# Autodesk Inventor assembly: outer_mirrored
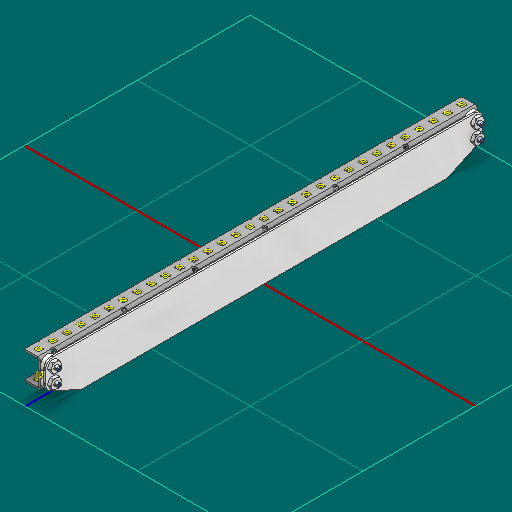
[picture p0: Inventor's stored thumbnail of the model, 512x512]
Saved by Autodesk Inventor 2025 (Build 290162000, 162)
## iProperties
Created: 2024-08-21
Part Number: outer_mirrored
Document SubType Name: Assembly
Designer: averey
Author: averey
## Documents named in this file (10)
- C:\Users\avere\vex_robotics_high_stakes\hardware\cad\bots\ENIGMA\chassis\drivetrain\drivebay_mirrored\outer_mirrored.iam
- C:\Users\avere\vex_robotics_high_stakes\hardware\cad\bots\ENIGMA\chassis\drivetrain\drivebay_mirrored\Alu C 1x2x1x31_mirrored.ipt
- C:\Users\avere\vex_robotics_high_stakes\hardware\cad\bots\ENIGMA\chassis\drivetrain\drivebay_mirrored\bearing_flat_w_hardware_mirrored.iam
- C:\Users\avere\vex_robotics_high_stakes\hardware\cad\VEX-CAD-Inventor\Motion\Spacers\Spacer Nylon .500 OD\NSpacer White .500 OD x .125.ipt
- C:\Users\avere\vex_robotics_high_stakes\hardware\cad\VEX-CAD-Inventor\Motion\Spacers\Spacer Nylon .500 OD.ipt
- C:\Users\avere\vex_robotics_high_stakes\hardware\cad\bots\ENIGMA\chassis\drivetrain\drivebay\custom_parts\skirt.ipt
- C:\Users\avere\vex_robotics_high_stakes\hardware\cad\VEX-CAD-Inventor\Structure\Hardware\Screw Shoulder Robosource\SScrew Shoulder Smooth .500 x .04.ipt
- C:\Users\avere\vex_robotics_high_stakes\hardware\cad\VEX-CAD-Inventor\Structure\Hardware\Screw Shoulder Robosource.ipt
- C:\Users\avere\vex_robotics_high_stakes\hardware\cad\VEX-CAD-Inventor\Structure\Hardware\Nut Nylon\Nut Nylon - White.ipt
- C:\Users\avere\vex_robotics_high_stakes\hardware\cad\VEX-CAD-Inventor\Structure\Hardware\Nut Nylon.ipt
## Components (23 placed, 6 different names)
1. Alu C 1x2x1x31_mirrored:1 — Mate:2, Mate:1, Mate:3, Insert:1, Insert:2, Insert:4
2. skirt:1 — Insert:3, Insert:5
3. bearing_flat_w_hardware_mirrored:1 [sub-assembly] — Mate:3, Insert:1
4. bearing_flat_w_hardware_mirrored:2 [sub-assembly]
5. bearing_flat_w_hardware_mirrored:3 [sub-assembly]
6. bearing_flat_w_hardware_mirrored:4 [sub-assembly]
7. bearing_flat_w_hardware_mirrored:5 [sub-assembly]
8. bearing_flat_w_hardware_mirrored:6 [sub-assembly]
9. bearing_flat_w_hardware_mirrored:7 [sub-assembly]
10. bearing_flat_w_hardware_mirrored:8 [sub-assembly]
11. bearing_flat_w_hardware_mirrored:9 [sub-assembly]
12. Nut Nylon - White:1 — Insert:5
13. SScrew Shoulder Smooth .500 x .04:1 — Insert:4
14. NSpacer White .500 OD x .125:1 — Insert:2, Insert:3
15. Nut Nylon - White:2
16. SScrew Shoulder Smooth .500 x .04:2
17. NSpacer White .500 OD x .125:2
18. Nut Nylon - White:3
19. SScrew Shoulder Smooth .500 x .04:3
20. NSpacer White .500 OD x .125:3
21. Nut Nylon - White:4
22. SScrew Shoulder Smooth .500 x .04:4
23. NSpacer White .500 OD x .125:4
## Component patterns: (9 elements, first: bearing_flat_w_hardware_mirrored:1), Hardware (4 elements)
## Relationships (8: Insert 5, Mate 3)
- Mate:2 (11.1125 mm): Alu C 1x2x1x31_mirrored:1
- Mate:1: Alu C 1x2x1x31_mirrored:1
- Mate:3: Alu C 1x2x1x31_mirrored:1 ↔ bearing_flat_w_hardware_mirrored:1
- Insert:1: Alu C 1x2x1x31_mirrored:1 ↔ bearing_flat_w_hardware_mirrored:1
- Insert:2: Alu C 1x2x1x31_mirrored:1 ↔ NSpacer White .500 OD x .125:1
- Insert:3: skirt:1 ↔ NSpacer White .500 OD x .125:1
- Insert:4: Alu C 1x2x1x31_mirrored:1 ↔ SScrew Shoulder Smooth .500 x .04:1
- Insert:5: skirt:1 ↔ Nut Nylon - White:1
